# Autodesk Inventor assembly: uniondosbaterias
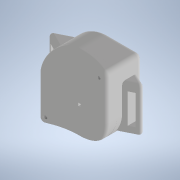
[picture p0: Inventor's stored thumbnail of the model, 180x180]
Saved by Autodesk Inventor 2020 (Build 240168000, 168)
## iProperties
Created: 2020-11-25
Part Number: uniondosbaterias
Document SubType Name: Assembly
Designer: itala
Author: itala
## Documents named in this file (9)
- C:\Users\itala\Google Drive (itala.latorre@pucp.edu.pe)\laptop2020\EEGGCC\2020-2\Fundamentos de biodiseño\dos baterias\uniondosbaterias.iam
- C:\Users\itala\Google Drive (itala.latorre@pucp.edu.pe)\laptop2020\EEGGCC\2020-2\Fundamentos de biodiseño\dos baterias\tapasuperiorbaterias2.ipt
- C:\Users\itala\Google Drive (itala.latorre@pucp.edu.pe)\laptop2020\EEGGCC\2020-2\Fundamentos de biodiseño\dos baterias\tapainferiorbaterias2.ipt
- C:\Users\itala\Google Drive (itala.latorre@pucp.edu.pe)\laptop2020\EEGGCC\2020-2\Fundamentos de biodiseño\Diseño 2\ASSEMBLY_AP214.iam
- C:\Users\itala\Google Drive (itala.latorre@pucp.edu.pe)\laptop2020\EEGGCC\2020-2\Fundamentos de biodiseño\Diseño 2\bateria litio.ipt
- C:\Users\itala\Google Drive (itala.latorre@pucp.edu.pe)\laptop2020\EEGGCC\2020-2\Fundamentos de biodiseño\Diseño 2\LM35-NOPB--3DModel-STEP-56544.ipt
- C:\Users\itala\Google Drive (itala.latorre@pucp.edu.pe)\laptop2020\EEGGCC\2020-2\Fundamentos de biodiseño\Diseño 2\OLED-128x64-0.96.ipt
- C:\Users\itala\Google Drive (itala.latorre@pucp.edu.pe)\laptop2020\EEGGCC\2020-2\Fundamentos de biodiseño\Diseño 2\SENSOR DE LA PULSERA.ipt
- C:\Users\itala\Google Drive (itala.latorre@pucp.edu.pe)\laptop2020\EEGGCC\2020-2\Fundamentos de biodiseño\Diseño 2\switch.ipt
## Components (9 placed, 8 different names)
1. tapasuperiorbaterias2:1 — Coincidencia:11, Coincidencia:12, Coincidencia:13, Coincidencia:14, Nivelación:3, Nivelación:4, Coincidencia:15, Nivelación:5, Nivelación:6
2. tapainferiorbaterias2:1 — Coincidencia:2, Coincidencia:3, Coincidencia:4, Insertar:1, Tangente:1, Coincidencia:6, Coincidencia:7, Coincidencia:8, Coincidencia:9, Coincidencia:10, Coincidencia:15, Nivelación:5, Nivelación:6
3. ASSEMBLY_AP214:1 [sub-assembly] — Coincidencia:5, Coincidencia:6, Coincidencia:7
4. bateria litio:1 — Coincidencia:1, Nivelación:1, Nivelación:2
5. LM35-NOPB--3DModel-STEP-56544:1 — Coincidencia:14, Nivelación:3, Nivelación:4
6. OLED-128x64-0.96:1 — Insertar:1, Tangente:1, Coincidencia:5
7. SENSOR DE LA PULSERA:1 — Coincidencia:11, Coincidencia:12, Coincidencia:13
8. switch:1 — Coincidencia:8, Coincidencia:9, Coincidencia:10
9. bateria litio:2 — Coincidencia:1, Nivelación:1, Nivelación:2, Coincidencia:2, Coincidencia:3, Coincidencia:4
## Relationships (23: Mate 15, Flush 6, Insert 1, Tangent 1)
- Coincidencia:1 [Mate]: bateria litio:1 ↔ bateria litio:2
- Nivelación:1 [Flush]: bateria litio:1 ↔ bateria litio:2
- Nivelación:2 [Flush]: bateria litio:1 ↔ bateria litio:2
- Coincidencia:2 [Mate]: tapainferiorbaterias2:1 ↔ bateria litio:2
- Coincidencia:3 [Mate]: tapainferiorbaterias2:1 ↔ bateria litio:2
- Coincidencia:4 [Mate]: tapainferiorbaterias2:1 ↔ bateria litio:2
- Insertar:1: tapainferiorbaterias2:1 ↔ OLED-128x64-0.96:1
- Tangente:1: tapainferiorbaterias2:1 ↔ OLED-128x64-0.96:1
- Coincidencia:5 [Mate]: ASSEMBLY_AP214:1 ↔ OLED-128x64-0.96:1
- Coincidencia:6 [Mate] (2 mm): tapainferiorbaterias2:1 ↔ ASSEMBLY_AP214:1
- Coincidencia:7 [Mate]: tapainferiorbaterias2:1 ↔ ASSEMBLY_AP214:1
- Coincidencia:8 [Mate]: tapainferiorbaterias2:1 ↔ switch:1
- Coincidencia:9 [Mate] (4 mm): tapainferiorbaterias2:1 ↔ switch:1
- Coincidencia:10 [Mate] (3 mm): tapainferiorbaterias2:1 ↔ switch:1
- Coincidencia:11 [Mate]: tapasuperiorbaterias2:1 ↔ SENSOR DE LA PULSERA:1
- Coincidencia:12 [Mate]: tapasuperiorbaterias2:1 ↔ SENSOR DE LA PULSERA:1
- Coincidencia:13 [Mate]: tapasuperiorbaterias2:1 ↔ SENSOR DE LA PULSERA:1
- Coincidencia:14 [Mate]: tapasuperiorbaterias2:1 ↔ LM35-NOPB--3DModel-STEP-56544:1
- Nivelación:3 [Flush] (5 mm): tapasuperiorbaterias2:1 ↔ LM35-NOPB--3DModel-STEP-56544:1
- Nivelación:4 [Flush] (8 mm): tapasuperiorbaterias2:1 ↔ LM35-NOPB--3DModel-STEP-56544:1
- Coincidencia:15 [Mate]: tapasuperiorbaterias2:1 ↔ tapainferiorbaterias2:1
- Nivelación:5 [Flush]: tapasuperiorbaterias2:1 ↔ tapainferiorbaterias2:1
- Nivelación:6 [Flush]: tapasuperiorbaterias2:1 ↔ tapainferiorbaterias2:1
